# Autodesk Inventor assembly: Coupler bottom to Xrail test
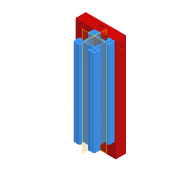
[picture p0: Inventor's stored thumbnail of the model, 180x180]
Saved by Autodesk Inventor 2020 (Build 240168000, 168)
## iProperties
Created: 2019-11-24
Part Number: Coupler bottom to Xrail test
Document SubType Name: Assembly
Designer: ball
Author: ball
## Documents named in this file (5)
- C:\FTC\FTC8863CAD\2019 Robot\Delivery\Coupler bottom to Xrail test.iam
- C:\FTC\FTC8863CAD\Actobotics\565 parts\565018.ipt
- C:\FTC\FTC8863CAD\2019 Robot\Delivery\Coupler top fixed front.ipt
- C:\FTC\FTC8863CAD\StepLibraries\Screws\6-32x.375_18-8 SS TRUSS HEAD PHILLIPS MACHINE SCREW.ipt
- C:\FTC\FTC8863CAD\Actobotics\585 parts\585757.ipt
## Components (5 placed, 4 different names)
1. 565018:1 — Mate:1, Flush:1, Flush:2, Flush:3, Mate:6
2. Coupler top fixed front:1 — Mate:1, Flush:1, Flush:2, Mate:2, Mate:3, Mate:4, Mate:5, Mate:7
3. 6-32x.375_18-8 SS TRUSS HEAD PHILLIPS MACHINE SCREW:1 — Mate:2, Mate:4
4. 6-32x.375_18-8 SS TRUSS HEAD PHILLIPS MACHINE SCREW:2 — Mate:3, Mate:5
5. 585757:1 — Flush:3, Mate:6, Mate:7
## Relationships (10: Mate 7, Flush 3)
- Mate:1: 565018:1 ↔ Coupler top fixed front:1
- Flush:1: 565018:1 ↔ Coupler top fixed front:1
- Flush:2: 565018:1 ↔ Coupler top fixed front:1
- Mate:2: Coupler top fixed front:1 ↔ 6-32x.375_18-8 SS TRUSS HEAD PHILLIPS MACHINE SCREW:1
- Mate:3: Coupler top fixed front:1 ↔ 6-32x.375_18-8 SS TRUSS HEAD PHILLIPS MACHINE SCREW:2
- Mate:4: Coupler top fixed front:1 ↔ 6-32x.375_18-8 SS TRUSS HEAD PHILLIPS MACHINE SCREW:1
- Mate:5: Coupler top fixed front:1 ↔ 6-32x.375_18-8 SS TRUSS HEAD PHILLIPS MACHINE SCREW:2
- Flush:3: 565018:1 ↔ 585757:1
- Mate:6: 565018:1 ↔ 585757:1
- Mate:7: Coupler top fixed front:1 ↔ 585757:1
